# Autodesk Inventor assembly: HK0609FM
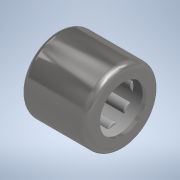
[picture p0: Inventor's stored thumbnail of the model, 180x180]
Saved by Autodesk Inventor 2021.3 (Build 253353000, 353)
## iProperties
Part Number: HK0609FM
Catalog Web Link: www.cadenas.de
Description: HK,HK..ZWD,HMK,HMK..ZWD (Open-end)-
Vendor: NTN
Document SubType Name: Assembly
Designer: partserver
Manufacturer: NTN
Mass: 0.324533 g
Surface Area: 12.6466 cm^2
Volume: 0.324533 cm^3
Density: 1 g/cm^3
Category: PARTsolutions
Company: NTN
PSOL_IDENT_0: {$CADENAS_DATA\23d-libs\ntn\needle_roler_bearings\needle_roller_shell_bearings\needle_roller_shell_b
PSOL_IDENT_1: earings_open_ended_asmtab.prj},198 {VTYP=3D},{STYP=ASSTAB},{NB=HK0609FM},{LINA=HK0609FM},{NN=HK,HK..
PSOL_IDENT_2: ZWD,HMK,HMK..ZWD (Open-end)},{DATE=23.10.2020 01:12:41},{GEOMDATE=22.04.2020 01:03:43},{VERSION=},{L
PSOL_IDENT_3: INEID=40},{WBVAR=},{WBNUMERIC=}  {NB=HK0609FM},{LINA=HK0609FM},{KT=DUMMY},{ORDER=HK0609FM},{FW=6},{D=
PSOL_IDENT_4: 10.0},{C=9},{CR=2920},{COR=2590},{CU=315},{CRF=298},{CORF=264},{LSG=25000},{LSO=37000},{MASS=0.0022}
PSOL_IDENT_5: ,{IT=-},{RT=1.6},{VER=1},{T=0.500},{DW=1.500},{LW=5.000},{NR=9.000},{CID=6.750},{CD=8.250},{CW=7.600
PSOL_IDENT_6: },{SD=6.300},{PPATH=../needle_roller_shell_bearings_open_ended_asmtpl.prj}
NB: HK0609FM
NN: HK,HK..ZWD,HMK,HMK..ZWD (Open-end)
NBSYN: $ORDER.
LINA: HK0609FM
CATALOG: NTN Corporation
ORDER: HK0609FM
FW: 6
D: 10
C: 9
CR: 2920
COR: 2590
CU: 315
LSG: 25000
LSO: 37000
MASS: 0.0022
IT: -
SUPPLIER: NTN
ARTICLENO: HK0609FM
BOMINFO: HK0609FM
CREATOR: CADENAS GmbH
Title: HK0609FM
Author: Cadenas PARTsolutions
## Documents named in this file (4)
- C:\Users\YusukeKunita\Documents\GrabCAD\NHK2021\BasicParts\よく使う部品（萩原）\Bearing\Bearing_HK0609FM\HK0609FM.iam
- C:\Users\YusukeKunita\Documents\GrabCAD\NHK2021\BasicParts\よく使う部品（萩原）\Bearing\Bearing_HK0609FM\HK0609FMSH.ipt
- C:\Users\YusukeKunita\Documents\GrabCAD\NHK2021\BasicParts\よく使う部品（萩原）\Bearing\Bearing_HK0609FM\HK0609FMCA.ipt
- C:\Users\YusukeKunita\Documents\GrabCAD\NHK2021\BasicParts\よく使う部品（萩原）\Bearing\Bearing_HK0609FM\HK0609FMRO.ipt
## Components (11 placed, 3 different names)
1. HK0609FMSH:1 — IP_5_XY@1 <-> IP_1_XY@2, IP_5_Z@1 <-> IP_1_Z@2
2. HK0609FMCA:1 — IP_5_XY@1 <-> IP_1_XY@2, IP_5_Z@1 <-> IP_1_Z@2, IP_3_1_XY@2 <-> IP_1_XY@3, IP_3_1_Z@2 <-> IP_1_Z@3, IP_3_1_YZ@2 <-> IP_1_YZ@3, IP_3_2_XY@2 <-> IP_1_XY@4, IP_3_2_Z@2 <-> IP_1_Z@4, IP_3_2_YZ@2 <-> IP_1_YZ@4, IP_3_3_XY@2 <-> IP_1_XY@5, IP_3_3_Z@2 <-> IP_1_Z@5, IP_3_3_YZ@2 <-> IP_1_YZ@5, IP_3_4_XY@2 <-> IP_1_XY@6, IP_3_4_Z@2 <-> IP_1_Z@6, IP_3_4_YZ@2 <-> IP_1_YZ@6, IP_3_5_XY@2 <-> IP_1_XY@7, IP_3_5_Z@2 <-> IP_1_Z@7, IP_3_5_YZ@2 <-> IP_1_YZ@7, IP_3_6_XY@2 <-> IP_1_XY@8, IP_3_6_Z@2 <-> IP_1_Z@8, IP_3_6_YZ@2 <-> IP_1_YZ@8, IP_3_7_XY@2 <-> IP_1_XY@9, IP_3_7_Z@2 <-> IP_1_Z@9, IP_3_7_YZ@2 <-> IP_1_YZ@9, IP_3_8_XY@2 <-> IP_1_XY@10, IP_3_8_Z@2 <-> IP_1_Z@10, IP_3_8_YZ@2 <-> IP_1_YZ@10, IP_3_9_XY@2 <-> IP_1_XY@11, IP_3_9_Z@2 <-> IP_1_Z@11, IP_3_9_YZ@2 <-> IP_1_YZ@11
3. HK0609FMRO:1 — IP_3_1_XY@2 <-> IP_1_XY@3, IP_3_1_Z@2 <-> IP_1_Z@3, IP_3_1_YZ@2 <-> IP_1_YZ@3
4. HK0609FMRO:2 — IP_3_2_XY@2 <-> IP_1_XY@4, IP_3_2_Z@2 <-> IP_1_Z@4, IP_3_2_YZ@2 <-> IP_1_YZ@4
5. HK0609FMRO:3 — IP_3_3_XY@2 <-> IP_1_XY@5, IP_3_3_Z@2 <-> IP_1_Z@5, IP_3_3_YZ@2 <-> IP_1_YZ@5
6. HK0609FMRO:4 — IP_3_4_XY@2 <-> IP_1_XY@6, IP_3_4_Z@2 <-> IP_1_Z@6, IP_3_4_YZ@2 <-> IP_1_YZ@6
7. HK0609FMRO:5 — IP_3_5_XY@2 <-> IP_1_XY@7, IP_3_5_Z@2 <-> IP_1_Z@7, IP_3_5_YZ@2 <-> IP_1_YZ@7
8. HK0609FMRO:6 — IP_3_6_XY@2 <-> IP_1_XY@8, IP_3_6_Z@2 <-> IP_1_Z@8, IP_3_6_YZ@2 <-> IP_1_YZ@8
9. HK0609FMRO:7 — IP_3_7_XY@2 <-> IP_1_XY@9, IP_3_7_Z@2 <-> IP_1_Z@9, IP_3_7_YZ@2 <-> IP_1_YZ@9
10. HK0609FMRO:8 — IP_3_8_XY@2 <-> IP_1_XY@10, IP_3_8_Z@2 <-> IP_1_Z@10, IP_3_8_YZ@2 <-> IP_1_YZ@10
11. HK0609FMRO:9 — IP_3_9_XY@2 <-> IP_1_XY@11, IP_3_9_Z@2 <-> IP_1_Z@11, IP_3_9_YZ@2 <-> IP_1_YZ@11
## Relationships (29: Mate 19, Angle 9, Flush 1)
- IP_5_XY@1 <-> IP_1_XY@2 [Flush]: HK0609FMSH:1 ↔ HK0609FMCA:1
- IP_5_Z@1 <-> IP_1_Z@2 [Mate]: HK0609FMSH:1 ↔ HK0609FMCA:1
- IP_3_1_XY@2 <-> IP_1_XY@3 [Mate]: HK0609FMCA:1 ↔ HK0609FMRO:1
- IP_3_1_Z@2 <-> IP_1_Z@3 [Mate]: HK0609FMCA:1 ↔ HK0609FMRO:1
- IP_3_1_YZ@2 <-> IP_1_YZ@3 [Angle] (0 deg): HK0609FMCA:1 ↔ HK0609FMRO:1
- IP_3_2_XY@2 <-> IP_1_XY@4 [Mate]: HK0609FMCA:1 ↔ HK0609FMRO:2
- IP_3_2_Z@2 <-> IP_1_Z@4 [Mate]: HK0609FMCA:1 ↔ HK0609FMRO:2
- IP_3_2_YZ@2 <-> IP_1_YZ@4 [Angle] (0 deg): HK0609FMCA:1 ↔ HK0609FMRO:2
- IP_3_3_XY@2 <-> IP_1_XY@5 [Mate]: HK0609FMCA:1 ↔ HK0609FMRO:3
- IP_3_3_Z@2 <-> IP_1_Z@5 [Mate]: HK0609FMCA:1 ↔ HK0609FMRO:3
- IP_3_3_YZ@2 <-> IP_1_YZ@5 [Angle] (0 deg): HK0609FMCA:1 ↔ HK0609FMRO:3
- IP_3_4_XY@2 <-> IP_1_XY@6 [Mate]: HK0609FMCA:1 ↔ HK0609FMRO:4
- IP_3_4_Z@2 <-> IP_1_Z@6 [Mate]: HK0609FMCA:1 ↔ HK0609FMRO:4
- IP_3_4_YZ@2 <-> IP_1_YZ@6 [Angle] (0 deg): HK0609FMCA:1 ↔ HK0609FMRO:4
- IP_3_5_XY@2 <-> IP_1_XY@7 [Mate]: HK0609FMCA:1 ↔ HK0609FMRO:5
- IP_3_5_Z@2 <-> IP_1_Z@7 [Mate]: HK0609FMCA:1 ↔ HK0609FMRO:5
- IP_3_5_YZ@2 <-> IP_1_YZ@7 [Angle] (0 deg): HK0609FMCA:1 ↔ HK0609FMRO:5
- IP_3_6_XY@2 <-> IP_1_XY@8 [Mate]: HK0609FMCA:1 ↔ HK0609FMRO:6
- IP_3_6_Z@2 <-> IP_1_Z@8 [Mate]: HK0609FMCA:1 ↔ HK0609FMRO:6
- IP_3_6_YZ@2 <-> IP_1_YZ@8 [Angle] (0 deg): HK0609FMCA:1 ↔ HK0609FMRO:6
- IP_3_7_XY@2 <-> IP_1_XY@9 [Mate]: HK0609FMCA:1 ↔ HK0609FMRO:7
- IP_3_7_Z@2 <-> IP_1_Z@9 [Mate]: HK0609FMCA:1 ↔ HK0609FMRO:7
- IP_3_7_YZ@2 <-> IP_1_YZ@9 [Angle] (0 deg): HK0609FMCA:1 ↔ HK0609FMRO:7
- IP_3_8_XY@2 <-> IP_1_XY@10 [Mate]: HK0609FMCA:1 ↔ HK0609FMRO:8
- IP_3_8_Z@2 <-> IP_1_Z@10 [Mate]: HK0609FMCA:1 ↔ HK0609FMRO:8
- IP_3_8_YZ@2 <-> IP_1_YZ@10 [Angle] (0 deg): HK0609FMCA:1 ↔ HK0609FMRO:8
- IP_3_9_XY@2 <-> IP_1_XY@11 [Mate]: HK0609FMCA:1 ↔ HK0609FMRO:9
- IP_3_9_Z@2 <-> IP_1_Z@11 [Mate]: HK0609FMCA:1 ↔ HK0609FMRO:9
- IP_3_9_YZ@2 <-> IP_1_YZ@11 [Angle] (0 deg): HK0609FMCA:1 ↔ HK0609FMRO:9
